# Autodesk Inventor assembly: main climber
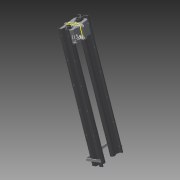
[picture p0: Inventor's stored thumbnail of the model, 180x180]
Saved by Autodesk Inventor 2013 (Build 170138000, 138)
## iProperties
Created: 2013-01-25
Part Number: main climber
Document SubType Name: Assembly
Designer: Arpan
Author: Arpan
## Documents named in this file (5)
- C:\Users\Arpan\Documents\GitHub\frc2013CAD\Cimber actual\main climber.iam
- C:\Users\Arpan\Documents\GitHub\frc2013CAD\Cimber actual\Shaft 26 inch.ipt
- C:\Users\Arpan\Documents\GitHub\frc2013CAD\Cimber actual\Bearing Block long style.iam
- C:\Users\Arpan\Documents\GitHub\frc2013CAD\Cimber actual\hook mount plate.ipt
- C:\Users\Arpan\Documents\GitHub\frc2013CAD\Cimber actual\tie-together tier 1.ipt
## Components (7 placed, 4 different names)
1. Shaft 26 inch:1 — Flush:1, Angle:1, Mate:2, Flush:2, Angle:2
2. Shaft 26 inch:2 — Flush:1, Angle:1, Mate:1, Flush:2, Mate:7, Mate:8, Mate:9
3. Bearing Block long style:1 [sub-assembly] — Mate:1, Mate:3, Flush:3, Mate:6, Flush:5
4. Bearing Block long style:2 [sub-assembly] — Mate:2, Mate:3, Angle:2, Flush:3, Mate:4, Flush:4, Mate:5
5. hook mount plate:1 — Mate:4, Flush:4, Mate:5, Flush:6
6. hook mount plate:2 — Mate:6, Flush:5, Flush:6
7. tie-together tier 1:1 — Mate:7, Mate:8, Mate:9
## Relationships (17: Mate 9, Flush 6, Angle 2)
- Flush:1: Shaft 26 inch:1 ↔ Shaft 26 inch:2
- Angle:1 (180 deg): Shaft 26 inch:1 ↔ Shaft 26 inch:2
- Mate:1: Shaft 26 inch:2 ↔ Bearing Block long style:1
- Mate:2: Shaft 26 inch:1 ↔ Bearing Block long style:2
- Mate:3 (12.7 mm): Bearing Block long style:1 ↔ Bearing Block long style:2
- Flush:2: Shaft 26 inch:1 ↔ Shaft 26 inch:2
- Angle:2 (0 deg): Shaft 26 inch:1 ↔ Bearing Block long style:2
- Flush:3: Bearing Block long style:1 ↔ Bearing Block long style:2
- Mate:4: Bearing Block long style:2 ↔ hook mount plate:1
- Flush:4: Bearing Block long style:2 ↔ hook mount plate:1
- Mate:5: Bearing Block long style:2 ↔ hook mount plate:1
- Mate:6: Bearing Block long style:1 ↔ hook mount plate:2
- Flush:5: Bearing Block long style:1 ↔ hook mount plate:2
- Flush:6: hook mount plate:1 ↔ hook mount plate:2
- Mate:7 (25.4 mm): Shaft 26 inch:2 ↔ tie-together tier 1:1
- Mate:8: Shaft 26 inch:2 ↔ tie-together tier 1:1
- Mate:9 (23.4188 mm): Shaft 26 inch:2 ↔ tie-together tier 1:1
